# Autodesk Inventor assembly: ASY МОО 001 отстойник осветлитель
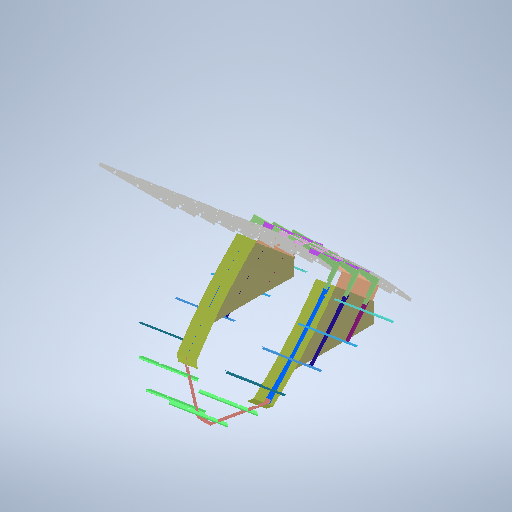
[picture p0: Inventor's stored thumbnail of the model, 512x512]
Saved by Autodesk Inventor 2025 (Build 290162010, 162A)
## iProperties
Created: 2024-04-28
Part Number: ASY МОО 001 отстойник осветлитель
Document SubType Name: Weldment
Designer: admin
Weld Material: Welded Aluminum-6061
Mass: 1.58517e+06 g
Surface Area: 1.48953e+06 cm^2
Volume: 226523 cm^3
Density: 6.99781 g/cm^3
Author: admin
## Documents named in this file (75)
- C:\Users\user\YandexDisk\домашниий пк\Inventor\Manturovo\Manturovo_Se-clar\ASY МОО 001 отстойник осветлитель.iam
- C:\Users\user\YandexDisk\домашниий пк\Inventor\Manturovo\Manturovo_Se-clar\MSC 033 sheet back basic.ipt
- C:\Users\user\YandexDisk\домашниий пк\Inventor\Manturovo\Manturovo_Se-clar\Пример емкости.ipt
- C:\Users\user\YandexDisk\домашниий пк\Inventor\Manturovo\Manturovo_Se-clar\MSC 041 sheet belly main.ipt
- C:\Users\user\YandexDisk\домашниий пк\Inventor\Manturovo\Manturovo_Se-clar\MSC 052 rib board.ipt
- C:\Users\user\YandexDisk\домашниий пк\Inventor\Manturovo\Manturovo_Se-clar\MSC 051 rib back.ipt
- C:\Users\user\YandexDisk\домашниий пк\Inventor\Manturovo\Manturovo_Se-clar\Рама основания\ASY MSC 090 base frame.iam
- C:\Users\user\YandexDisk\домашниий пк\Inventor\Manturovo\Manturovo_Se-clar\ASY MSC 080 roсket.iam
- C:\Users\user\YandexDisk\домашниий пк\Inventor\Manturovo\Manturovo_Se-clar\ASY MSC 010 cone.iam
- C:\Users\user\YandexDisk\домашниий пк\Inventor\Manturovo\Manturovo_Se-clar\ракета\МОО 064 ракета труба.ipt
- C:\Users\user\YandexDisk\домашниий пк\Inventor\Manturovo\Manturovo_Se-clar\MSC 000 DIM settler-clarifier.ipt
- C:\Users\user\YandexDisk\домашниий пк\Inventor\Manturovo\Manturovo_Se-clar\MSC 031 sheet lowerback.ipt
- C:\Users\user\YandexDisk\домашниий пк\Inventor\Manturovo\Manturovo_Se-clar\MSC 024 sheet board main.ipt
- C:\Users\user\YandexDisk\домашниий пк\Inventor\Manturovo\Manturovo_Se-clar\MSC 032 sheet magic back-lowerback.ipt
- C:\Users\user\YandexDisk\домашниий пк\Inventor\Manturovo\Manturovo_Se-clar\MSC 021 sheet left board hip.ipt
- C:\Users\user\YandexDisk\домашниий пк\Inventor\Manturovo\Manturovo_Se-clar\MSC 022 sheet right board hip.ipt
- C:\Users\user\YandexDisk\домашниий пк\Inventor\Manturovo\Manturovo_Se-clar\MSC 034 sheet back-neck.ipt
- C:\Users\user\YandexDisk\домашниий пк\Inventor\Manturovo\Manturovo_Se-clar\MSC 042 sheet belly-neck.ipt
- C:\Users\user\YandexDisk\домашниий пк\Inventor\Manturovo\Manturovo_Se-clar\MSC 023 sheet board.ipt
- C:\Users\user\YandexDisk\домашниий пк\Inventor\Manturovo\Manturovo_Se-clar\конус\MSC 071 ridge 1.ipt
- C:\Users\user\YandexDisk\домашниий пк\Inventor\Manturovo\Manturovo_Se-clar\конус\MSC 073 ridge 3.ipt
- C:\Users\user\YandexDisk\домашниий пк\Inventor\Manturovo\Manturovo_Se-clar\конус\MSC 074 face 1.ipt
- C:\Users\user\YandexDisk\домашниий пк\Inventor\Manturovo\Manturovo_Se-clar\Content Center Files\en-US\ISO 5251 B 3D\ISO 5251 Bends 3D without straight ends(90 deg) DN150 11 11.ipt
- C:\Users\user\YandexDisk\домашниий пк\Inventor\Manturovo\Manturovo_Se-clar\Content Center Files\en-US\DIN EN 1092-1 01 - PN 25\DIN EN 1092-1 Plate Flange for Welding Type 01 - PN 25 150 x 168.3.ipt
- C:\Users\user\YandexDisk\домашниий пк\Inventor\Manturovo\Manturovo_Se-clar\МОО 061 труба верх 1.ipt
- C:\Users\user\YandexDisk\домашниий пк\Inventor\Manturovo\Manturovo_Se-clar\МОО 062 труба верх 2.ipt
- C:\Users\user\YandexDisk\домашниий пк\Inventor\Manturovo\Manturovo_Se-clar\МОО 063 труба верх 3.ipt
- C:\Users\user\YandexDisk\домашниий пк\Inventor\Manturovo\Manturovo_Se-clar\MSC 061 stringer back ^.ipt
- C:\Users\user\YandexDisk\домашниий пк\Inventor\Manturovo\Manturovo_Se-clar\MSC 063 stringer board #.ipt
- C:\Users\user\YandexDisk\домашниий пк\Inventor\Manturovo\Manturovo_Se-clar\MSC 062 stringer back ^^.ipt
- C:\Users\user\YandexDisk\домашниий пк\Inventor\Manturovo\Manturovo_Se-clar\MSC 064 stringer board ##.ipt
- C:\Users\user\YandexDisk\домашниий пк\Inventor\Manturovo\Manturovo_Se-clar\MSC 065 stringer board ###.ipt
- C:\Users\user\YandexDisk\домашниий пк\Inventor\Manturovo\Manturovo_Se-clar\MSC 066 stringer board ####.ipt
- C:\Users\user\YandexDisk\домашниий пк\Inventor\Manturovo\Manturovo_Se-clar\MSC 067 stringer board belly.ipt
- C:\Users\user\YandexDisk\домашниий пк\Inventor\Manturovo\Manturovo_Se-clar\MSC 053 rib belly.ipt
- C:\Users\user\YandexDisk\домашниий пк\Inventor\Manturovo\Manturovo_Se-clar\MSC 025 sheet board withers 1.ipt
- C:\Users\user\YandexDisk\домашниий пк\Inventor\Manturovo\Manturovo_Se-clar\MSC 027 sheet board face 1.ipt
- C:\Users\user\YandexDisk\домашниий пк\Inventor\Manturovo\Manturovo_Se-clar\Part1.ipt
- C:\Users\user\YandexDisk\домашниий пк\Inventor\Manturovo\Manturovo_Se-clar\стапель\ASY стапель.iam
- C:\Users\user\YandexDisk\домашниий пк\Inventor\Manturovo\Manturovo_Se-clar\MSC 0101 sheet gills.ipt
- C:\Users\user\YandexDisk\домашниий пк\Inventor\Manturovo\Manturovo_Se-clar\MSC 026 sheet board withers 2.ipt
- C:\Users\user\YandexDisk\домашниий пк\Inventor\Manturovo\Manturovo_Se-clar\MSC 028 sheet board face 2.ipt
- C:\Users\user\YandexDisk\домашниий пк\Inventor\Manturovo\Manturovo_Se-clar\MSC 068 stringer lowerback.ipt
- C:\Users\user\YandexDisk\домашниий пк\Inventor\Manturovo\Manturovo_Se-clar\конус\MSC 072 ridge 2.ipt
- C:\Users\user\YandexDisk\домашниий пк\Inventor\Manturovo\Manturovo_Se-clar\MSC 075 face 2.ipt
- C:\Users\user\YandexDisk\домашниий пк\Inventor\Manturovo\Manturovo_Se-clar\MSC 076 face 3.ipt
- C:\Users\user\YandexDisk\домашниий пк\Inventor\Manturovo\Manturovo_Se-clar\MSC 077 face 4.ipt
- C:\Users\user\YandexDisk\домашниий пк\Inventor\Manturovo\Manturovo_Se-clar\MSC 055 rib hip 2.ipt
- C:\Users\user\YandexDisk\домашниий пк\Inventor\Manturovo\Manturovo_Se-clar\MSC 110 revision hatch 1.ipt
- C:\Users\user\YandexDisk\домашниий пк\Inventor\Manturovo\Manturovo_Se-clar\MSC 054 rib hip 1.ipt
- C:\Users\user\YandexDisk\домашниий пк\Inventor\Manturovo\Manturovo_Se-clar\MSC 035 ring.ipt
- C:\Users\user\YandexDisk\домашниий пк\Inventor\Manturovo\Manturovo_Se-clar\MSC 074 ridge 4.ipt
- C:\Users\user\YandexDisk\домашниий пк\Inventor\Manturovo\Manturovo_Se-clar\MSC 075 ridge 5.ipt
- C:\Users\user\YandexDisk\домашниий пк\Inventor\Manturovo\Manturovo_Se-clar\MSC 081 pillar 1.ipt
- C:\Users\user\YandexDisk\домашниий пк\Inventor\Manturovo\Manturovo_Se-clar\MSC 036 flange 500.ipt
- C:\Users\user\YandexDisk\домашниий пк\Inventor\Manturovo\Manturovo_Se-clar\MSC 037 flange cover 500.ipt
- C:\Users\user\YandexDisk\домашниий пк\Inventor\Manturovo\Manturovo_Se-clar\MSC 038 flange cover ring 500.ipt
- C:\Users\user\YandexDisk\домашниий пк\Inventor\Manturovo\Manturovo_Se-clar\MSC 039 flange cover plate 500.ipt
- C:\Users\user\YandexDisk\домашниий пк\Inventor\Manturovo\Manturovo_Se-clar\Content Center Files\en-US\DIN EN ISO 8676\DIN EN ISO 8676 - M12 x 1,5 x 30.ipt
- C:\Users\user\YandexDisk\домашниий пк\Inventor\Manturovo\Manturovo_Se-clar\Content Center Files\en-US\ISO 4032(2)\ISO 4032 - M12 - ISO.ipt
- C:\Users\user\YandexDisk\домашниий пк\Inventor\Manturovo\Manturovo_Se-clar\Рама основания\ASY MSC 120  base frame.iam
- C:\Users\user\YandexDisk\домашниий пк\Inventor\Manturovo\Manturovo_Se-clar\Рама основания\ASY MSC 121  base frame.iam
- C:\Users\user\YandexDisk\домашниий пк\Inventor\Manturovo\Manturovo_Se-clar\Чертеж для парам. рамы.ipt
- C:\Users\user\YandexDisk\домашниий пк\Inventor\Manturovo\Manturovo_Se-clar\ASY MSC 120.1  base frame.iam
- C:\Users\user\YandexDisk\домашниий пк\Inventor\Manturovo\Manturovo_Se-clar\ASY MSC 122  base frame.iam
- C:\Users\user\YandexDisk\домашниий пк\Inventor\Manturovo\Manturovo_Se-clar\ASY MSC 123  base frame.iam
- C:\Users\user\YandexDisk\домашниий пк\Inventor\Manturovo\Manturovo_Se-clar\ASY MSC 124  base frame.iam
- C:\Users\user\YandexDisk\домашниий пк\Inventor\Manturovo\Manturovo_Se-clar\MSC 125 base tube.ipt
- C:\Users\user\YandexDisk\домашниий пк\Inventor\Manturovo\Manturovo_Se-clar\MSC 126 flange base tube.ipt
- C:\Users\user\YandexDisk\домашниий пк\Inventor\Manturovo\Manturovo_Se-clar\MSC 128 flange base tube support.ipt
- C:\Users\user\YandexDisk\домашниий пк\Inventor\Manturovo\Manturovo_Se-clar\MSC 125 base tube_MIR2.ipt
- C:\Users\user\YandexDisk\домашниий пк\Inventor\Manturovo\Manturovo_Se-clar\DXF файлы\MSC 126 flange base tube_MIR2.ipt
- C:\Users\user\YandexDisk\домашниий пк\Inventor\Manturovo\Manturovo_Se-clar\DXF файлы\MSC 128 flange base tube support_MIR1.ipt
- C:\Users\user\YandexDisk\домашниий пк\Inventor\Manturovo\Manturovo_Se-clar\MSC 0331 sheet back mould.ipt
- C:\Users\user\YandexDisk\домашниий пк\Inventor\Manturovo\Manturovo_Se-clar\MSC 0511 rib back mould.ipt
## Components (298 placed, 82 different names)
1. Пример емкости.ipt:1 — Mate:1, Mate:2, Flush:2
2. MSC 000 DIM settler-clarifier.ipt:1
3. ASY MSC 090 base frame.iam:1 [sub-assembly] — Flush:19, Flush:21, Flush:82, Mate:82
4. ASY MSC 010 cone.iam:1 [sub-assembly] — Flush:22, Mate:16, Flush:28, Mate:31, Mate:36, Mate:54, Mate:57, Mate:65, Mate:78, Tangent:11, Flush:79, Mate:82, Mate:83
5. MSC 033 sheet back basic.ipt:1 — Flush:3, Rigid:11, Rigid:12
6. MSC 041 sheet belly main.ipt:1 — Mate:9, Rigid:18, Rigid:40
7. ASY MSC 080 roсket.iam:1 [sub-assembly] — Flush:23
8. МОО 064 ракета труба.ipt:1
9. MSC 033 sheet back basic.ipt:2 — Rigid:11, Tangent:1, Tangent:3, Rigid:37
10. MSC 033 sheet back basic.ipt:3 — Flush:24, Rigid:12, Mate:19, Mate:22, Rigid:30, Mate:31, Flush:44, Tangent:8, Tangent:9
11. MSC 031 sheet lowerback.ipt:1 — Mate:15, Mate:16, Mate:19, Mate:22, Tangent:10, Tangent:11, Tangent:12, Cylindrical:2
12. MSC 024 sheet board main.ipt:1 — Flush:30, Tangent:1, Rigid:35, Mate:37
13. MSC 041 sheet belly main.ipt:2 — Rigid:18, Rigid:53
14. MSC 032 sheet magic back-lowerback.ipt:1 — Mate:24, Rigid:30, Flush:42, Tangent:6, Flush:43, Tangent:7
15. MSC 021 sheet left board hip.ipt:1 — Flush:41, Flush:42, Tangent:6, Mate:78
16. MSC 022 sheet right board hip.ipt:1 — Mate:30, Flush:43, Tangent:7
17. MSC 024 sheet board main.ipt:2 — Rigid:35, Rigid:36
18. MSC 024 sheet board main.ipt:3 — Rigid:36, Rigid:49
19. MSC 033 sheet back basic.ipt:4 — Rigid:37, Rigid:38
20. MSC 033 sheet back basic.ipt:5 — Rigid:38, Rigid:39, Tangent:14
21. MSC 034 sheet back-neck.ipt:1 — Rigid:39
22. MSC 041 sheet belly main.ipt:3 — Rigid:40, Rigid:47
23. MSC 042 sheet belly-neck.ipt:1 — Rigid:48, Mate:70, Mate:71
24. MSC 041 sheet belly main.ipt:4 — Rigid:45, Rigid:47
25. MSC 041 sheet belly main.ipt:5 — Rigid:45, Rigid:48
26. MSC 024 sheet board main.ipt:4 — Rigid:49, Rigid:50
27. MSC 024 sheet board main.ipt:5 — Rigid:50, Rigid:113
28. MSC 023 sheet board.ipt:1 — Mate:36, Flush:47, Tangent:8, Mate:37, Mate:55
29. MSC 071 ridge 1.ipt:1 — Mate:50, Flush:57, Mate:68, Flush:81, Flush:83, Mate:85
30. MSC 074 face 1.ipt:1 — Rigid:156, Rigid:157, Mate:70, Flush:62, Mate:71, Rigid:159, Mate:80
31. MSC 041 sheet belly main.ipt:6 — Mate:54, Mate:55, Rigid:53, Mate:93, Mate:96
32. MSC 073 ridge 3.ipt:1 — Flush:56, Flush:57, Mate:68, Mate:77, Flush:78, Mate:81, Flush:80
33. DIN EN 1092-1 Plate Flange for Welding Type 01 - PN 25 150 x 168.3.ipt:1 — Rigid:158
34. МОО 061 труба верх 1.ipt:1 — Rigid:158, Rigid:59, Rigid:159
35. ISO 5251 Bends 3D without straight ends(90 deg) DN150 11 11.ipt:1 — Rigid:59, Rotational:2
36. МОО 062 труба верх 2.ipt:1 — Rigid:132, Rigid:156
37. DIN EN 1092-1 Plate Flange for Welding Type 01 - PN 25 150 x 168.3.ipt:2 — Rigid:132
38. МОО 063 труба верх 3.ipt:1 — Rigid:157
39. MSC 024 sheet board main.ipt:6 — Rigid:134
40. MSC 024 sheet board main.ipt:7
41. MSC 024 sheet board main.ipt:8
42. MSC 024 sheet board main.ipt:9
43. MSC 024 sheet board main.ipt:10 — Rigid:67
44. MSC 023 sheet board.ipt:2 — Rigid:67, Mate:57, Mate:58, Tangent:9
45. MSC 052 rib board.ipt:1 — Rigid:74, Rigid:161, Rigid:162, Rigid:163, Rigid:164
46. MSC 051 rib back.ipt:1 — Rigid:25, Rigid:74, Rigid:91, Rigid:93, Rigid:139
47. MSC 066 stringer board ####.ipt:1 — Rigid:143, Rigid:162
48. MSC 065 stringer board ###.ipt:1 — Rigid:142, Rigid:163
49. MSC 064 stringer board ##.ipt:1 — Rigid:141, Rigid:164
50. MSC 063 stringer board #.ipt:1 — Rigid:140
51. MSC 062 stringer back ^^.ipt:1 — Rigid:93, Rigid:155, Mate:84
52. MSC 061 stringer back ^.ipt:2 — Rigid:91, Rigid:153
53. MSC 061 stringer back ^.ipt:1 — Rigid:90, Rigid:152
54. MSC 025 sheet board withers 1.ipt:1 — Rigid:113, Rigid:114
55. MSC 027 sheet board face 1.ipt:1 — Rigid:114, Flush:56, Mate:69, Flush:60, Mate:75
56. Part1.ipt:1
57. MSC 051 rib back.ipt:2 — Rigid:116, Rigid:130, Rigid:131, Rigid:169
58. MSC 051 rib back.ipt:3 — Rigid:116, Rigid:171
59. MSC 051 rib back.ipt:4 — Rigid:131, Rigid:170
60. MSC 051 rib back.ipt:5 — Mate:62, Flush:53, Rigid:172
61. MSC 062 stringer back ^^.ipt:2 — Rigid:92, Mate:66, Rigid:154
62. MSC 066 stringer board ####.ipt:2 — Rigid:125, Rigid:151
63. MSC 063 stringer board #.ipt:2 — Rigid:148
64. MSC 064 stringer board ##.ipt:2 — Rigid:149, Rigid:167
65. MSC 065 stringer board ###.ipt:2 — Rigid:150, Rigid:166
66. MSC 052 rib board.ipt:3 — Rigid:72, Flush:51, Flush:52, Rigid:125, Mate:61, Rigid:166, Rigid:167, Rigid:168
67. MSC 051 rib back.ipt:6 — Flush:12, Tangent:3, Rigid:25, Flush:44, Rigid:72, Rigid:90, Rigid:92, Rigid:130
68. ASY стапель.iam:1 [sub-assembly] — Mate:62, Flush:53, Mate:63
69. MSC 053 rib belly.ipt:2 — Rigid:110, Flush:51, Flush:52, Rigid:126, Mate:61, Rigid:127
70. MSC 053 rib belly.ipt:1 — Rigid:111, Rigid:112, Rigid:127
71. MSC 067 stringer board belly.ipt:4 — Rigid:126, Rigid:147
72. MSC 067 stringer board belly.ipt:3 — Rigid:110, Rigid:146
73. MSC 067 stringer board belly.ipt:2 — Rigid:112, Rigid:144
74. MSC 067 stringer board belly.ipt:1 — Rigid:111, Rigid:145
75. MSC 0101 sheet gills.ipt:1 — Mate:64
76. MSC 026 sheet board withers 2.ipt:1 — Rigid:133, Rigid:134
77. MSC 028 sheet board face 2.ipt:1 — Rigid:133
78. MSC 068 stringer lowerback.ipt:1 — Mate:65, Mate:66, Tangent:10
79. MSC 072 ridge 2.ipt:1 — Flush:58, Mate:81, Flush:80, Flush:81, Flush:84
80. МОО 061 труба верх 1.ipt:2 — Rotational:2
81. MSC 075 face 2.ipt:1 — Mate:69, Flush:60, Flush:61, Mate:76
82. MSC 076 face 3.ipt:1 — Flush:76, Mate:75, Mate:76
83. MSC 077 face 4.ipt:1 — Mate:77, Flush:77, Flush:78, Mate:80
84. MSC 055 rib hip 2:1 — Rigid:169
85. MSC 110 revision hatch 1:1 — Flush:82
86. MSC 054 rib board hip 1:1 — Rigid:170
87. MSC 055 rib hip 2:2 — Rigid:171
88. MSC 054 rib board hip 1:2 — Rigid:172
89. MSC 068 stringer lowerback:2 — Mate:83, Mate:84, Tangent:12
90. MSC 035 ring:1 — Rotational:3, Cylindrical:2
91. MSC 074 ridge 4:1 — Flush:83, Mate:85, Flush:84, Rigid:173
92. MSC 075 ridge 5:1 — Rigid:173
93. MSC 081 pillar 1:1 — Insert:1, Insert:2, Insert:3, Insert:4, Rigid:179, Mate:93
94. MSC 036 flange 500:1 — Rigid:175
95. MSC 036 flange 500:2 — Rigid:175, Rigid:176
96. MSC 036 flange 500:3 — Rigid:176, Rigid:177, Rotational:3, Mate:87
97. MSC 036 flange 500:4 — Rigid:177, Rotational:4
98. MSC 037 flange cover 500:1 — Rotational:4, Mate:87, Rigid:178, Mate:89
99. MSC 038 flange cover ring 500:1 — Rigid:178, Tangent:13
100. DIN EN ISO 8676 M12 x 1,5 x 30:1 — Rigid:179
101. ISO 4032 M12:1 — Insert:2
102. ISO 4032 M12:2 — Insert:1
103. ISO 4032 M12:3 — Insert:3
104. ISO 4032 M12:4 — Insert:4
105. ASY MSC 120  base frame:1 [sub-assembly] — Flush:93, Mate:97, Rotational:5
106. ASY MSC 121  base frame:1 [sub-assembly] — Mate:98, Flush:95, Mate:99
107. Чертеж для парам. рамы:1 — Flush:94, Mate:95, Mate:96, Mate:97, Mate:99, Mate:100, Mate:103, Mate:105, Mate:107
108. ASY MSC 120.1  base frame:2 [sub-assembly] — Flush:96, Mate:100, Mate:101
109. ASY MSC 122  base frame:2 [sub-assembly] — Flush:97, Mate:102, Mate:103
110. ASY MSC 123  base frame:2 [sub-assembly] — Flush:98, Mate:104, Mate:105
111. ASY MSC 124  base frame:2 [sub-assembly] — Flush:99, Mate:106, Mate:107
112. MSC 0511 rib back mould:1
113. MSC 053 rib belly.ipt:3
114. MSC 052 rib board.ipt:4
115. MSC 051 rib back.ipt:7 — Rigid:139
116. MSC 051 rib back.ipt:8
117. MSC 052 rib board.ipt:5
118. MSC 053 rib belly.ipt:4
119. MSC 053 rib belly.ipt:5
120. MSC 052 rib board.ipt:6
121. MSC 051 rib back.ipt:9
122. MSC 051 rib back.ipt:10
123. MSC 052 rib board.ipt:7
124. MSC 053 rib belly.ipt:6
125. MSC 053 rib belly.ipt:7
126. MSC 052 rib board.ipt:8
127. MSC 051 rib back.ipt:11
128. MSC 051 rib back.ipt:12
129. MSC 052 rib board.ipt:9
130. MSC 053 rib belly.ipt:8
131. MSC 053 rib belly.ipt:9
132. MSC 052 rib board.ipt:10
133. MSC 051 rib back.ipt:13
134. MSC 051 rib back.ipt:14
135. MSC 052 rib board.ipt:11
136. MSC 053 rib belly.ipt:10
137. MSC 053 rib belly.ipt:11
138. MSC 052 rib board.ipt:12
139. MSC 051 rib back.ipt:15
140. MSC 051 rib back.ipt:16
141. MSC 052 rib board.ipt:13
142. MSC 053 rib belly.ipt:12
143. MSC 053 rib belly.ipt:13
144. MSC 052 rib board.ipt:14
145. MSC 051 rib back.ipt:17
146. MSC 051 rib back.ipt:18
147. MSC 052 rib board.ipt:15
148. MSC 053 rib belly.ipt:14
149. MSC 053 rib belly.ipt:15
150. MSC 052 rib board.ipt:16
151. MSC 051 rib back.ipt:19
152. MSC 051 rib back.ipt:20
153. MSC 052 rib board.ipt:17
154. MSC 053 rib belly.ipt:16
155. MSC 053 rib belly.ipt:17
156. MSC 052 rib board.ipt:18
157. MSC 051 rib back.ipt:21
158. MSC 051 rib back.ipt:22
159. MSC 052 rib board.ipt:19
160. MSC 053 rib belly.ipt:18
161. MSC 053 rib belly.ipt:19
162. MSC 052 rib board.ipt:20
163. MSC 051 rib back.ipt:23
164. MSC 051 rib back.ipt:24
165. MSC 052 rib board.ipt:21
166. MSC 053 rib belly.ipt:20
167. MSC 053 rib belly.ipt:21
168. MSC 052 rib board.ipt:22
169. MSC 051 rib back.ipt:25
170. MSC 051 rib back.ipt:26
171. MSC 052 rib board.ipt:23
172. MSC 053 rib belly.ipt:22
173. MSC 053 rib belly.ipt:23
174. MSC 052 rib board.ipt:24
175. MSC 051 rib back.ipt:27
176. MSC 051 rib back.ipt:28
177. MSC 052 rib board.ipt:25
178. MSC 053 rib belly.ipt:24
179. MSC 053 rib belly.ipt:25
180. MSC 052 rib board.ipt:26
181. MSC 051 rib back.ipt:29
182. MSC 051 rib back.ipt:30
183. MSC 052 rib board.ipt:27
184. MSC 053 rib belly.ipt:26
185. MSC 063 stringer board #.ipt:3 — Rigid:148, Rigid:168
186. MSC 064 stringer board ##.ipt:3 — Rigid:149
187. MSC 065 stringer board ###.ipt:3 — Rigid:150
188. MSC 066 stringer board ####.ipt:3 — Rigid:151
189. MSC 067 stringer board belly.ipt:5 — Rigid:147
190. MSC 067 stringer board belly.ipt:6 — Rigid:146
191. MSC 062 stringer back ^^.ipt:3 — Rigid:154
192. MSC 061 stringer back ^.ipt:3 — Rigid:152
193. MSC 061 stringer back ^.ipt:4 — Rigid:153
194. MSC 062 stringer back ^^.ipt:4 — Rigid:155
195. MSC 063 stringer board #.ipt:4 — Rigid:140, Rigid:161
196. MSC 064 stringer board ##.ipt:4 — Rigid:141
197. MSC 065 stringer board ###.ipt:4 — Rigid:142
198. MSC 066 stringer board ####.ipt:4 — Rigid:143
199. MSC 067 stringer board belly.ipt:7 — Rigid:145
200. MSC 067 stringer board belly.ipt:8 — Rigid:144
201. MSC 063 stringer board #.ipt:5
202. MSC 064 stringer board ##.ipt:5
203. MSC 065 stringer board ###.ipt:5
204. MSC 066 stringer board ####.ipt:5
205. MSC 067 stringer board belly.ipt:9
206. MSC 067 stringer board belly.ipt:10
207. MSC 062 stringer back ^^.ipt:5
208. MSC 061 stringer back ^.ipt:5
209. MSC 061 stringer back ^.ipt:6
210. MSC 062 stringer back ^^.ipt:6
211. MSC 063 stringer board #.ipt:6
212. MSC 064 stringer board ##.ipt:6
213. MSC 065 stringer board ###.ipt:6
214. MSC 066 stringer board ####.ipt:6
215. MSC 067 stringer board belly.ipt:11
216. MSC 067 stringer board belly.ipt:12
217. MSC 063 stringer board #.ipt:7
218. MSC 064 stringer board ##.ipt:7
219. MSC 065 stringer board ###.ipt:7
220. MSC 066 stringer board ####.ipt:7
221. MSC 067 stringer board belly.ipt:13
222. MSC 067 stringer board belly.ipt:14
223. MSC 062 stringer back ^^.ipt:7
224. MSC 061 stringer back ^.ipt:7
225. MSC 061 stringer back ^.ipt:8
226. MSC 062 stringer back ^^.ipt:8
227. MSC 063 stringer board #.ipt:8
228. MSC 064 stringer board ##.ipt:8
229. MSC 065 stringer board ###.ipt:8
230. MSC 066 stringer board ####.ipt:8
231. MSC 067 stringer board belly.ipt:15
232. MSC 067 stringer board belly.ipt:16
233. МОО 053 стрингер борт 3:9
234. МОО 054 стрингер борт 4:9
235. МОО 055 стрингер борт 5:9
236. МОО 056 стрингер борт 6:10
237. МОО 057 стрингер борт 7:19
238. МОО 057 стрингер борт 7:20
239. МОО 052 стрингер спина 2:9
240. МОО 051 стрингер спина 1:9
241. МОО 051 стрингер спина 1:10
242. МОО 052 стрингер спина 2:10
243. МОО 053 стрингер борт 3:10
244. МОО 054 стрингер борт 4:10
245. МОО 055 стрингер борт 5:10
246. МОО 056 стрингер борт 6:11
247. МОО 057 стрингер борт 7:21
248. МОО 057 стрингер борт 7:22
249. MSC 039 flange cover plate 500:1 — Tangent:13, Mate:89
250. MSC 039 flange cover plate 500:2
251. MSC 039 flange cover plate 500:3
252. MSC 039 flange cover plate 500:4
253. MSC 039 flange cover plate 500:5
254. MSC 039 flange cover plate 500:6
255. MSC 039 flange cover plate 500:7
256. MSC 039 flange cover plate 500:8
257. MSC 039 flange cover plate 500:9
258. MSC 039 flange cover plate 500:10
259. MSC 039 flange cover plate 500:11
260. MSC 039 flange cover plate 500:12
261. MSC 126 flange base tube_MIR2:1 — Rigid:183
262. MSC 125 base tube_MIR2:1 — Rigid:183, Rigid:184
263. MSC 128 flange base tube support_MIR1:1 — Rigid:184
264. MSC 125 base tube:1 — Rigid:180, Rigid:182
265. MSC 128 flange base tube support:1 — Rigid:182
266. MSC 126 flange base tube:1 — Rigid:180, Rotational:5
267. MSC 126 flange base tube_MIR2:2
268. MSC 125 base tube_MIR2:2
269. MSC 128 flange base tube support_MIR1:2
270. MSC 125 base tube:2
271. MSC 128 flange base tube support:2
272. MSC 126 flange base tube:2
273. MSC 126 flange base tube_MIR2:3
274. MSC 125 base tube_MIR2:3
275. MSC 128 flange base tube support_MIR1:3
276. MSC 125 base tube:3
277. MSC 128 flange base tube support:3
278. MSC 126 flange base tube:3
279. MSC 126 flange base tube_MIR2:4
280. MSC 125 base tube_MIR2:4
281. MSC 128 flange base tube support_MIR1:4
282. MSC 125 base tube:4
283. MSC 128 flange base tube support:4
284. MSC 126 flange base tube:4
285. MSC 0331 sheet back mould:1 — Tangent:14, Flush:100
286. MSC 0331 sheet back mould:2
287. MSC 0331 sheet back mould:3
288. MSC 0331 sheet back mould:4
289. MSC 0331 sheet back mould:5
290. MSC 0331 sheet back mould:6
291. MSC 0331 sheet back mould:7
292. MSC 0331 sheet back mould:8
293. MSC 0331 sheet back mould:9
294. MSC 0331 sheet back mould:10
295. MSC 0331 sheet back mould:11
296. MSC 0331 sheet back mould:12
297. MSC 0331 sheet back mould:13
298. MSC 0331 sheet back mould:14
## Component patterns: (12 elements, first: MSC 053 rib belly.ipt:3 + MSC 052 rib board.ipt:4 + MSC 051 rib back.ipt:7 + MSC 051 rib back.ipt:8 + MSC 052 rib board.ipt:5 + MSC 053 rib belly.ipt:4), (4 elements, first: MSC 063 stringer board #.ipt:3 + MSC 064 stringer board ##.ipt:3 + MSC 065 stringer board ###.ipt:3 + MSC 066 stringer board ####.ipt:3 + MSC 067 stringer board belly.ipt:5 + MSC 067 stringer board belly.ipt:6 + MSC 062 stringer back ^^.ipt:3 + MSC 061 stringer back ^.ipt:3 + MSC 061 stringer back ^.ipt:4 + MSC 062 stringer back ^^.ipt:4 + MSC 063 stringer board #.ipt:4 + MSC 064 stringer board ##.ipt:4 + MSC 065 stringer board ###.ipt:4 + MSC 066 stringer board ####.ipt:4 + MSC 067 stringer board belly.ipt:7 + MSC 067 stringer board belly.ipt:8), (12 elements, first: MSC 039 flange cover plate 500:1), (4 elements, first: MSC 126 flange base tube_MIR2:1 + MSC 125 base tube_MIR2:1 + MSC 128 flange base tube support_MIR1:1 + MSC 125 base tube:1 + MSC 128 flange base tube support:1 + MSC 126 flange base tube:1), (14 elements, first: MSC 0331 sheet back mould:1)
## Relationships (208: WeldJoint 90, Mate 55, Flush 43, Tangent 11, RevoluteJoint 4, Insert 4, CylindricalJoint 1)
- Mate:1: Пример емкости.ipt:1
- Mate:2: Пример емкости.ipt:1
- Flush:2: Пример емкости.ipt:1
- Flush:3: MSC 033 sheet back basic.ipt:1
- Mate:9: MSC 041 sheet belly main.ipt:1
- Flush:12: MSC 051 rib back.ipt:6
- Flush:19: ASY MSC 090 base frame.iam:1
- Flush:21: ASY MSC 090 base frame.iam:1
- Flush:22: ASY MSC 010 cone.iam:1
- Flush:23: ASY MSC 080 roсket.iam:1
- Mate:15: MSC 031 sheet lowerback.ipt:1
- Flush:24: MSC 033 sheet back basic.ipt:3
- Mate:16: ASY MSC 010 cone.iam:1 ↔ MSC 031 sheet lowerback.ipt:1
- Flush:28: ASY MSC 010 cone.iam:1
- Rigid:11 [WeldJoint]: MSC 033 sheet back basic.ipt:1 ↔ MSC 033 sheet back basic.ipt:2
- Rigid:12 [WeldJoint]: MSC 033 sheet back basic.ipt:1 ↔ MSC 033 sheet back basic.ipt:3
- Mate:19 (910 mm): MSC 033 sheet back basic.ipt:3 ↔ MSC 031 sheet lowerback.ipt:1
- Flush:30: MSC 024 sheet board main.ipt:1
- Tangent:1: MSC 033 sheet back basic.ipt:2 ↔ MSC 024 sheet board main.ipt:1
- Tangent:3: MSC 033 sheet back basic.ipt:2 ↔ MSC 051 rib back.ipt:6
- Mate:22 (47 mm): MSC 033 sheet back basic.ipt:3 ↔ MSC 031 sheet lowerback.ipt:1
- Rigid:18 [WeldJoint]: MSC 041 sheet belly main.ipt:1 ↔ MSC 041 sheet belly main.ipt:2
- Rigid:25 [WeldJoint] (-50 mm): MSC 051 rib back.ipt:1 ↔ MSC 051 rib back.ipt:6
- Mate:24: MSC 032 sheet magic back-lowerback.ipt:1
- Rigid:30 [WeldJoint]: MSC 033 sheet back basic.ipt:3 ↔ MSC 032 sheet magic back-lowerback.ipt:1
- Flush:41: MSC 021 sheet left board hip.ipt:1
- Flush:42: MSC 032 sheet magic back-lowerback.ipt:1 ↔ MSC 021 sheet left board hip.ipt:1
- Tangent:6: MSC 032 sheet magic back-lowerback.ipt:1 ↔ MSC 021 sheet left board hip.ipt:1
- Mate:30: MSC 022 sheet right board hip.ipt:1
- Flush:43: MSC 032 sheet magic back-lowerback.ipt:1 ↔ MSC 022 sheet right board hip.ipt:1
- Tangent:7: MSC 032 sheet magic back-lowerback.ipt:1 ↔ MSC 022 sheet right board hip.ipt:1
- Rigid:35 [WeldJoint]: MSC 024 sheet board main.ipt:1 ↔ MSC 024 sheet board main.ipt:2
- Rigid:36 [WeldJoint]: MSC 024 sheet board main.ipt:2 ↔ MSC 024 sheet board main.ipt:3
- Rigid:37 [WeldJoint]: MSC 033 sheet back basic.ipt:2 ↔ MSC 033 sheet back basic.ipt:4
- Rigid:38 [WeldJoint]: MSC 033 sheet back basic.ipt:4 ↔ MSC 033 sheet back basic.ipt:5
- Rigid:39 [WeldJoint]: MSC 033 sheet back basic.ipt:5 ↔ MSC 034 sheet back-neck.ipt:1
- Mate:31: ASY MSC 010 cone.iam:1 ↔ MSC 033 sheet back basic.ipt:3
- Rigid:40 [WeldJoint]: MSC 041 sheet belly main.ipt:1 ↔ MSC 041 sheet belly main.ipt:3
- Flush:44 (-250 mm): MSC 033 sheet back basic.ipt:3 ↔ MSC 051 rib back.ipt:6
- Rigid:45 [WeldJoint]: MSC 041 sheet belly main.ipt:4 ↔ MSC 041 sheet belly main.ipt:5
- Rigid:47 [WeldJoint]: MSC 041 sheet belly main.ipt:3 ↔ MSC 041 sheet belly main.ipt:4
- Rigid:48 [WeldJoint]: MSC 042 sheet belly-neck.ipt:1 ↔ MSC 041 sheet belly main.ipt:5
- Rigid:49 [WeldJoint]: MSC 024 sheet board main.ipt:3 ↔ MSC 024 sheet board main.ipt:4
- Rigid:50 [WeldJoint]: MSC 024 sheet board main.ipt:4 ↔ MSC 024 sheet board main.ipt:5
- Mate:36: ASY MSC 010 cone.iam:1 ↔ MSC 023 sheet board.ipt:1
- Flush:47: MSC 023 sheet board.ipt:1
- Tangent:8: MSC 033 sheet back basic.ipt:3 ↔ MSC 023 sheet board.ipt:1
- Mate:37: MSC 024 sheet board main.ipt:1 ↔ MSC 023 sheet board.ipt:1
- Mate:50 (200 mm): MSC 071 ridge 1.ipt:1
- Mate:54: ASY MSC 010 cone.iam:1 ↔ MSC 041 sheet belly main.ipt:6
- Mate:55: MSC 023 sheet board.ipt:1 ↔ MSC 041 sheet belly main.ipt:6
- Rigid:53 [WeldJoint]: MSC 041 sheet belly main.ipt:2 ↔ MSC 041 sheet belly main.ipt:6
- Rigid:158 [WeldJoint]: DIN EN 1092-1 Plate Flange for Welding Type 01 - PN 25 150 x 168.3.ipt:1 ↔ МОО 061 труба верх 1.ipt:1
- Rigid:59 [WeldJoint]: МОО 061 труба верх 1.ipt:1 ↔ ISO 5251 Bends 3D without straight ends(90 deg) DN150 11 11.ipt:1
- [WeldJoint]: MSC 024 sheet board main.ipt:6 ↔ MSC 024 sheet board main.ipt:7
- [WeldJoint]: MSC 024 sheet board main.ipt:7 ↔ MSC 024 sheet board main.ipt:8
- [WeldJoint]: MSC 024 sheet board main.ipt:8 ↔ MSC 024 sheet board main.ipt:9
- [WeldJoint]: MSC 024 sheet board main.ipt:9 ↔ MSC 024 sheet board main.ipt:10
- Rigid:67 [WeldJoint]: MSC 024 sheet board main.ipt:10 ↔ MSC 023 sheet board.ipt:2
- Mate:57: ASY MSC 010 cone.iam:1 ↔ MSC 023 sheet board.ipt:2
- Mate:58: MSC 023 sheet board.ipt:2
- Tangent:9: MSC 033 sheet back basic.ipt:3 ↔ MSC 023 sheet board.ipt:2
- Rigid:72 [WeldJoint] (-50 mm): MSC 052 rib board.ipt:3 ↔ MSC 051 rib back.ipt:6
- Rigid:74 [WeldJoint] (-50 mm): MSC 052 rib board.ipt:1 ↔ MSC 051 rib back.ipt:1
- Rigid:90 [WeldJoint] (2 mm): MSC 061 stringer back ^.ipt:1 ↔ MSC 051 rib back.ipt:6
- Rigid:91 [WeldJoint] (2 mm): MSC 051 rib back.ipt:1 ↔ MSC 061 stringer back ^.ipt:2
- Rigid:92 [WeldJoint] (2 mm): MSC 062 stringer back ^^.ipt:2 ↔ MSC 051 rib back.ipt:6
- Rigid:93 [WeldJoint] (2 mm): MSC 051 rib back.ipt:1 ↔ MSC 062 stringer back ^^.ipt:1
- Rigid:110 [WeldJoint] (2 mm): MSC 053 rib belly.ipt:2 ↔ MSC 067 stringer board belly.ipt:3
- Rigid:111 [WeldJoint] (2 mm): MSC 053 rib belly.ipt:1 ↔ MSC 067 stringer board belly.ipt:1
- Rigid:112 [WeldJoint] (2 mm): MSC 053 rib belly.ipt:1 ↔ MSC 067 stringer board belly.ipt:2
- Rigid:113 [WeldJoint]: MSC 024 sheet board main.ipt:5 ↔ MSC 025 sheet board withers 1.ipt:1
- Rigid:114 [WeldJoint]: MSC 025 sheet board withers 1.ipt:1 ↔ MSC 027 sheet board face 1.ipt:1
- Rigid:116 [WeldJoint] (50 mm): MSC 051 rib back.ipt:2 ↔ MSC 051 rib back.ipt:3
- [WeldJoint] (50 mm): MSC 051 rib back.ipt:4 ↔ MSC 051 rib back.ipt:5
- Flush:51: MSC 052 rib board.ipt:3 ↔ MSC 053 rib belly.ipt:2
- Flush:52: MSC 052 rib board.ipt:3 ↔ MSC 053 rib belly.ipt:2
- Rigid:125 [WeldJoint] (2 mm): MSC 066 stringer board ####.ipt:2 ↔ MSC 052 rib board.ipt:3
- Rigid:126 [WeldJoint] (2 mm): MSC 053 rib belly.ipt:2 ↔ MSC 067 stringer board belly.ipt:4
- Mate:61: MSC 052 rib board.ipt:3 ↔ MSC 053 rib belly.ipt:2
- Mate:62: MSC 051 rib back.ipt:5 ↔ ASY стапель.iam:1
- Flush:53: MSC 051 rib back.ipt:5 ↔ ASY стапель.iam:1
- Mate:63: ASY стапель.iam:1
- Rigid:127 [WeldJoint] (-50 mm): MSC 053 rib belly.ipt:2 ↔ MSC 053 rib belly.ipt:1
- Rigid:130 [WeldJoint] (-500 mm): MSC 051 rib back.ipt:2 ↔ MSC 051 rib back.ipt:6
- Rigid:131 [WeldJoint] (-500 mm): MSC 051 rib back.ipt:2 ↔ MSC 051 rib back.ipt:4
- Rigid:132 [WeldJoint]: МОО 062 труба верх 2.ipt:1 ↔ DIN EN 1092-1 Plate Flange for Welding Type 01 - PN 25 150 x 168.3.ipt:2
- Mate:64: MSC 0101 sheet gills.ipt:1
- Rigid:133 [WeldJoint]: MSC 026 sheet board withers 2.ipt:1 ↔ MSC 028 sheet board face 2.ipt:1
- Rigid:134 [WeldJoint]: MSC 024 sheet board main.ipt:6 ↔ MSC 026 sheet board withers 2.ipt:1
- Mate:65: ASY MSC 010 cone.iam:1 ↔ MSC 068 stringer lowerback.ipt:1
- Mate:66: MSC 062 stringer back ^^.ipt:2 ↔ MSC 068 stringer lowerback.ipt:1
- Tangent:10: MSC 031 sheet lowerback.ipt:1 ↔ MSC 068 stringer lowerback.ipt:1
- [WeldJoint] (-50 mm): MSC 051 rib back.ipt:7 ↔ MSC 051 rib back.ipt:8
- [WeldJoint] (-50 mm): MSC 051 rib back.ipt:8 ↔ MSC 052 rib board.ipt:5
- [WeldJoint] (-50 mm): MSC 052 rib board.ipt:4 ↔ MSC 051 rib back.ipt:7
- [Flush]: MSC 052 rib board.ipt:5 ↔ MSC 053 rib belly.ipt:4
- [Flush]: MSC 052 rib board.ipt:5 ↔ MSC 053 rib belly.ipt:4
- [Mate]: MSC 052 rib board.ipt:5 ↔ MSC 053 rib belly.ipt:4
- [WeldJoint] (-50 mm): MSC 053 rib belly.ipt:3 ↔ MSC 053 rib belly.ipt:4
- Rigid:139 [WeldJoint] (-500 mm): MSC 051 rib back.ipt:1 ↔ MSC 051 rib back.ipt:7
- Rigid:140 [WeldJoint] (2 mm): MSC 063 stringer board #.ipt:1 ↔ MSC 063 stringer board #.ipt:4
- Rigid:141 [WeldJoint]: MSC 064 stringer board ##.ipt:1 ↔ MSC 064 stringer board ##.ipt:4
- Rigid:142 [WeldJoint]: MSC 065 stringer board ###.ipt:1 ↔ MSC 065 stringer board ###.ipt:4
- Rigid:143 [WeldJoint]: MSC 066 stringer board ####.ipt:1 ↔ MSC 066 stringer board ####.ipt:4
- Rigid:144 [WeldJoint]: MSC 067 stringer board belly.ipt:2 ↔ MSC 067 stringer board belly.ipt:8
- Rigid:145 [WeldJoint]: MSC 067 stringer board belly.ipt:1 ↔ MSC 067 stringer board belly.ipt:7
- Rigid:146 [WeldJoint]: MSC 067 stringer board belly.ipt:3 ↔ MSC 067 stringer board belly.ipt:6
- Rigid:147 [WeldJoint]: MSC 067 stringer board belly.ipt:4 ↔ MSC 067 stringer board belly.ipt:5
- Rigid:148 [WeldJoint]: MSC 063 stringer board #.ipt:2 ↔ MSC 063 stringer board #.ipt:3
- Rigid:149 [WeldJoint]: MSC 064 stringer board ##.ipt:2 ↔ MSC 064 stringer board ##.ipt:3
- Rigid:150 [WeldJoint]: MSC 065 stringer board ###.ipt:2 ↔ MSC 065 stringer board ###.ipt:3
- Rigid:151 [WeldJoint]: MSC 066 stringer board ####.ipt:2 ↔ MSC 066 stringer board ####.ipt:3
- Rigid:152 [WeldJoint]: MSC 061 stringer back ^.ipt:1 ↔ MSC 061 stringer back ^.ipt:3
- Rigid:153 [WeldJoint]: MSC 061 stringer back ^.ipt:2 ↔ MSC 061 stringer back ^.ipt:4
- Rigid:154 [WeldJoint]: MSC 062 stringer back ^^.ipt:2 ↔ MSC 062 stringer back ^^.ipt:3
- Rigid:155 [WeldJoint]: MSC 062 stringer back ^^.ipt:1 ↔ MSC 062 stringer back ^^.ipt:4
- Flush:56 (200 mm): MSC 073 ridge 3.ipt:1 ↔ MSC 027 sheet board face 1.ipt:1
- Flush:57: MSC 071 ridge 1.ipt:1 ↔ MSC 073 ridge 3.ipt:1
- Mate:68: MSC 071 ridge 1.ipt:1 ↔ MSC 073 ridge 3.ipt:1
- Flush:58 (200 mm): MSC 072 ridge 2.ipt:1
- Rotational:2 [RevoluteJoint]: ISO 5251 Bends 3D without straight ends(90 deg) DN150 11 11.ipt:1 ↔ МОО 061 труба верх 1.ipt:2
- Mate:69: MSC 027 sheet board face 1.ipt:1 ↔ MSC 075 face 2.ipt:1
- Flush:60: MSC 027 sheet board face 1.ipt:1 ↔ MSC 075 face 2.ipt:1
- Flush:61: MSC 075 face 2.ipt:1
- Rigid:156 [WeldJoint]: MSC 074 face 1.ipt:1 ↔ МОО 062 труба верх 2.ipt:1
- Rigid:157 [WeldJoint]: MSC 074 face 1.ipt:1 ↔ МОО 063 труба верх 3.ipt:1
- Mate:70: MSC 042 sheet belly-neck.ipt:1 ↔ MSC 074 face 1.ipt:1
- Flush:62: MSC 074 face 1.ipt:1
- Mate:71: MSC 042 sheet belly-neck.ipt:1 ↔ MSC 074 face 1.ipt:1
- Rigid:159 [WeldJoint] (-200 mm): MSC 074 face 1.ipt:1 ↔ МОО 061 труба верх 1.ipt:1
- Flush:76: MSC 076 face 3.ipt:1
- Mate:75: MSC 027 sheet board face 1.ipt:1 ↔ MSC 076 face 3.ipt:1
- Mate:76: MSC 075 face 2.ipt:1 ↔ MSC 076 face 3.ipt:1
- Mate:77: MSC 073 ridge 3.ipt:1 ↔ MSC 077 face 4.ipt:1
- Flush:77: MSC 077 face 4.ipt:1
- Flush:78: MSC 073 ridge 3.ipt:1 ↔ MSC 077 face 4.ipt:1
- Mate:78: ASY MSC 010 cone.iam:1 ↔ MSC 021 sheet left board hip.ipt:1
- Tangent:11 (30 mm): ASY MSC 010 cone.iam:1 ↔ MSC 031 sheet lowerback.ipt:1
- Flush:79: ASY MSC 010 cone.iam:1
- Rigid:161 [WeldJoint] (2 mm): MSC 052 rib board.ipt:1 ↔ MSC 063 stringer board #.ipt:4
- Rigid:162 [WeldJoint] (2 mm): MSC 052 rib board.ipt:1 ↔ MSC 066 stringer board ####.ipt:1
- Rigid:163 [WeldJoint] (2 mm): MSC 052 rib board.ipt:1 ↔ MSC 065 stringer board ###.ipt:1
- Rigid:164 [WeldJoint] (2 mm): MSC 052 rib board.ipt:1 ↔ MSC 064 stringer board ##.ipt:1
- Mate:80: MSC 074 face 1.ipt:1 ↔ MSC 077 face 4.ipt:1
- Mate:81: MSC 073 ridge 3.ipt:1 ↔ MSC 072 ridge 2.ipt:1
- Flush:80: MSC 073 ridge 3.ipt:1 ↔ MSC 072 ridge 2.ipt:1
- Flush:81: MSC 071 ridge 1.ipt:1 ↔ MSC 072 ridge 2.ipt:1
- Rigid:166 [WeldJoint] (2 mm): MSC 065 stringer board ###.ipt:2 ↔ MSC 052 rib board.ipt:3
- Rigid:167 [WeldJoint] (2 mm): MSC 064 stringer board ##.ipt:2 ↔ MSC 052 rib board.ipt:3
- Rigid:168 [WeldJoint] (2 mm): MSC 052 rib board.ipt:3 ↔ MSC 063 stringer board #.ipt:3
- Rigid:169 [WeldJoint] (-50 mm): MSC 051 rib back.ipt:2 ↔ MSC 055 rib hip 2:1
- Flush:82: ASY MSC 090 base frame.iam:1 ↔ MSC 110 revision hatch 1:1
- Mate:82: ASY MSC 090 base frame.iam:1 ↔ ASY MSC 010 cone.iam:1
- Rigid:170 [WeldJoint] (-50 mm): MSC 051 rib back.ipt:4 ↔ MSC 054 rib board hip 1:1
- Rigid:171 [WeldJoint] (-50 mm): MSC 051 rib back.ipt:3 ↔ MSC 055 rib hip 2:2
- Rigid:172 [WeldJoint] (-50 mm): MSC 051 rib back.ipt:5 ↔ MSC 054 rib board hip 1:2
- Mate:83: ASY MSC 010 cone.iam:1 ↔ MSC 068 stringer lowerback:2
- Mate:84: MSC 062 stringer back ^^.ipt:1 ↔ MSC 068 stringer lowerback:2
- Tangent:12: MSC 031 sheet lowerback.ipt:1 ↔ MSC 068 stringer lowerback:2
- Flush:83: MSC 071 ridge 1.ipt:1 ↔ MSC 074 ridge 4:1
- Mate:85: MSC 071 ridge 1.ipt:1 ↔ MSC 074 ridge 4:1
- Flush:84: MSC 072 ridge 2.ipt:1 ↔ MSC 074 ridge 4:1
- Rigid:173 [WeldJoint]: MSC 074 ridge 4:1 ↔ MSC 075 ridge 5:1
- Rigid:175 [WeldJoint]: MSC 036 flange 500:1 ↔ MSC 036 flange 500:2
- Rigid:176 [WeldJoint]: MSC 036 flange 500:2 ↔ MSC 036 flange 500:3
- Rigid:177 [WeldJoint]: MSC 036 flange 500:3 ↔ MSC 036 flange 500:4
- Rotational:3 [RevoluteJoint]: MSC 035 ring:1 ↔ MSC 036 flange 500:3
- Cylindrical:2: MSC 031 sheet lowerback.ipt:1 ↔ MSC 035 ring:1
- Rotational:4 [RevoluteJoint]: MSC 036 flange 500:4 ↔ MSC 037 flange cover 500:1
- Mate:87: MSC 036 flange 500:3 ↔ MSC 037 flange cover 500:1
- Rigid:178 [WeldJoint]: MSC 037 flange cover 500:1 ↔ MSC 038 flange cover ring 500:1
- Tangent:13: MSC 038 flange cover ring 500:1 ↔ MSC 039 flange cover plate 500:1
- Mate:89: MSC 037 flange cover 500:1 ↔ MSC 039 flange cover plate 500:1
- Insert:1: MSC 081 pillar 1:1 ↔ ISO 4032 M12:2
- Insert:2: MSC 081 pillar 1:1 ↔ ISO 4032 M12:1
- Insert:3: MSC 081 pillar 1:1 ↔ ISO 4032 M12:3
- Insert:4: MSC 081 pillar 1:1 ↔ ISO 4032 M12:4
- Rigid:179 [WeldJoint] (-3 mm): MSC 081 pillar 1:1 ↔ DIN EN ISO 8676 M12 x 1,5 x 30:1
- Flush:93 (-3 mm): ASY MSC 120  base frame:1
- [Mate]: ASY MSC 120  base frame:1
- Mate:93: MSC 041 sheet belly main.ipt:6 ↔ MSC 081 pillar 1:1
- Flush:94: Чертеж для парам. рамы:1
- Mate:95: Чертеж для парам. рамы:1
- Mate:96: MSC 041 sheet belly main.ipt:6 ↔ Чертеж для парам. рамы:1
- Mate:97: ASY MSC 120  base frame:1 ↔ Чертеж для парам. рамы:1
- Mate:98: ASY MSC 121  base frame:1
- Flush:95 (-3 mm): ASY MSC 121  base frame:1
- Mate:99: ASY MSC 121  base frame:1 ↔ Чертеж для парам. рамы:1
- Flush:96 (-3 mm): ASY MSC 120.1  base frame:2
- Mate:100: Чертеж для парам. рамы:1 ↔ ASY MSC 120.1  base frame:2
- Mate:101: ASY MSC 120.1  base frame:2
- Flush:97 (-3 mm): ASY MSC 122  base frame:2
- Mate:102: ASY MSC 122  base frame:2
- Mate:103: Чертеж для парам. рамы:1 ↔ ASY MSC 122  base frame:2
- Flush:98 (-3 mm): ASY MSC 123  base frame:2
- Mate:104: ASY MSC 123  base frame:2
- Mate:105: Чертеж для парам. рамы:1 ↔ ASY MSC 123  base frame:2
- Flush:99 (-3 mm): ASY MSC 124  base frame:2
- Mate:106: ASY MSC 124  base frame:2
- Mate:107: Чертеж для парам. рамы:1 ↔ ASY MSC 124  base frame:2
- Rigid:180 [WeldJoint]: MSC 125 base tube:1 ↔ MSC 126 flange base tube:1
- Rotational:5 [RevoluteJoint]: ASY MSC 120  base frame:1 ↔ MSC 126 flange base tube:1
- Rigid:182 [WeldJoint]: MSC 125 base tube:1 ↔ MSC 128 flange base tube support:1
- Rigid:183 [WeldJoint]: MSC 126 flange base tube_MIR2:1 ↔ MSC 125 base tube_MIR2:1
- Rigid:184 [WeldJoint]: MSC 125 base tube_MIR2:1 ↔ MSC 128 flange base tube support_MIR1:1
- Tangent:14: MSC 033 sheet back basic.ipt:5 ↔ MSC 0331 sheet back mould:1
- Flush:100: MSC 0331 sheet back mould:1
## Named parameters: Бак_нахлест_фланца = 25 mm, d230_d194 = 0 mm, d231_d195 = 0 mm, d232_d160 = 0 mm, d233_d161 = 0 mm, d322_d320 = 50 mm, d384_d346 = 0 mm, d385_d359 = -50 mm, d386_d341 = 0 mm, d387_d342 = 0 mm, d388_d243 = -50 mm, d389_d246 = -50 mm, d390_d128 = -50 mm, Шаг_опор_по_баку = 2000 mm
